# Autodesk Inventor assembly: PitchingMachine
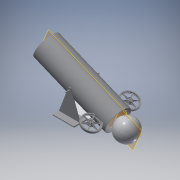
[picture p0: Inventor's stored thumbnail of the model, 180x180]
Saved by Autodesk Inventor 2016 SP1 (Build 200210100, 210)
## iProperties
Created: 2016-01-12
Part Number: PitchingMachine
Document SubType Name: Assembly
Designer: steele
Author: steele
## Documents named in this file (6)
- C:\snobotics\CAD-Development\robSteele\SnoBotics2016\FirstCutPitchingMachine\PitchingMachine.iam
- C:\snobotics\CAD-Development\robSteele\SnoBotics2016\FirstCutPitchingMachine\PitchingMachineBase.ipt
- C:\snobotics\CAD-Development\robSteele\SnoBotics2016\FirstCutPitchingMachine\PitchingMachineSupport.ipt
- C:\snobotics\CAD-Development\robSteele\SnoBotics2016\FirstCutPitchingMachine\pitchingMachineTube.ipt
- C:\snobotics\CAD-Development\robSteele\SnoBotics2016\FirstCutPitchingMachine\8 in Wheel\x2010-8-FIRSTwheel-375bear.ipt
- C:\snobotics\CAD-Development\robSteele\SnoBotics2016\DraftOfBoulder.ipt
## Components (7 placed, 5 different names)
1. PitchingMachineBase:1 — Mate:1, Flush:1, Mate:2, Mate:3, Flush:2, Mate:4
2. PitchingMachineSupport:1 — Mate:1, Flush:1, Mate:2, Insert:1
3. PitchingMachineSupport:2 — Mate:3, Flush:2, Mate:4
4. pitchingMachineTube:1 — Insert:1, Mate:5, Mate:8, Mate:9, Mate:10, Mate:11, Flush:3, Flush:4
5. x2010-8-FIRSTwheel-375bear:1 — Mate:5, Mate:6, Mate:8
6. x2010-8-FIRSTwheel-375bear:2 — Mate:9, Mate:10, Mate:11
7. DraftOfBoulder:1 — Flush:3, Flush:4
## Relationships (15: Mate 10, Flush 4, Insert 1)
- Mate:1: PitchingMachineBase:1 ↔ PitchingMachineSupport:1
- Flush:1: PitchingMachineBase:1 ↔ PitchingMachineSupport:1
- Mate:2: PitchingMachineBase:1 ↔ PitchingMachineSupport:1
- Mate:3: PitchingMachineBase:1 ↔ PitchingMachineSupport:2
- Flush:2: PitchingMachineBase:1 ↔ PitchingMachineSupport:2
- Mate:4: PitchingMachineBase:1 ↔ PitchingMachineSupport:2
- Insert:1: PitchingMachineSupport:1 ↔ pitchingMachineTube:1
- Mate:5: pitchingMachineTube:1 ↔ x2010-8-FIRSTwheel-375bear:1
- Mate:6 (228.6 mm): x2010-8-FIRSTwheel-375bear:1
- Mate:8: pitchingMachineTube:1 ↔ x2010-8-FIRSTwheel-375bear:1
- Mate:9: pitchingMachineTube:1 ↔ x2010-8-FIRSTwheel-375bear:2
- Mate:10 (-228.6 mm): pitchingMachineTube:1 ↔ x2010-8-FIRSTwheel-375bear:2
- Mate:11: pitchingMachineTube:1 ↔ x2010-8-FIRSTwheel-375bear:2
- Flush:3: pitchingMachineTube:1 ↔ DraftOfBoulder:1
- Flush:4: pitchingMachineTube:1 ↔ DraftOfBoulder:1
## Named parameters: pMSupportDistanceFromEdge = 127 mm
